# Autodesk Inventor assembly: main'
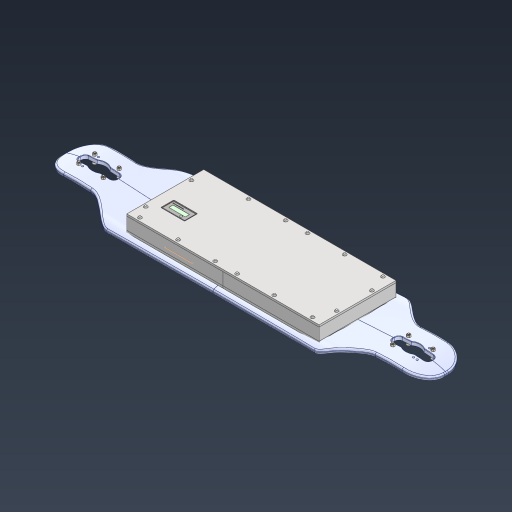
[picture p0: Inventor's stored thumbnail of the model, 512x512]
Saved by Autodesk Inventor 2023 (Build 270158000, 158)
## iProperties
Created: 2025-11-13
Part Number: main'
Document SubType Name: Assembly
Designer: szymo
Author: szymo
## iProperties of the stored document PG7 CABLE GLAND.ipt
Created: 2025-06-09
Part Number: PG7 CABLE GLAND
Material: Generic
Description: STEP AP214
Document SubType Name: Modeling
Designer: szymo
Density: 1 g/cm^3
Appearance: Default
Sending System: SolidWorks 2024
Preprocessor: SwSTEP 2.0
Title: PG7 CABLE GLAND.STEP
Revision Number: ANY
## Documents named in this file (32)
- D:\tech\diy\e-skateboard\projekcik-inventor\main.iam
- D:\tech\diy\e-skateboard\projekcik-inventor\mini-pakiet-12sp1.iam
- D:\tech\diy\e-skateboard\projekcik-inventor\6384 Motor.ipt
- D:\tech\diy\e-skateboard\projekcik-inventor\longboard\Longboard FreeRide.iam
- D:\tech\diy\e-skateboard\projekcik-inventor\vesc42.ipt
- D:\tech\diy\e-skateboard\projekcik-inventor\xt90.iam
- D:\tech\diy\e-skateboard\projekcik-inventor\buttoj\16mm-LED-Power-Button.iam
- **D:\tech\diy\e-skateboard\projekcik-inventor\main.iam*LocalDocs*xAaaaaxaaAaaaaaaaAaaaq0hoRf*PG7 CABLE GLAND.ipt
- D:\tech\diy\e-skateboard\projekcik-inventor\other-parts\deseczka_dol_check - 7.ipt
- D:\tech\diy\e-skateboard\projekcik-inventor\fuse.iam
- D:\tech\diy\e-skateboard\projekcik-inventor\led_buck_conv.ipt
- D:\tech\diy\e-skateboard\projekcik-inventor\battery_status_monitor.iam
- D:\tech\diy\e-skateboard\projekcik-inventor\MKS_express.ipt
- D:\tech\diy\e-skateboard\projekcik-inventor\controller_reveiver.ipt
- D:\tech\diy\e-skateboard\projekcik-inventor\buck_holder.ipt
- D:\tech\diy\e-skateboard\projekcik-inventor\vesc_holder.ipt
- D:\tech\diy\e-skateboard\projekcik-inventor\my_own_pcb.ipt
- D:\tech\diy\e-skateboard\projekcik-inventor\my_pcb_holder.ipt
- D:\tech\diy\e-skateboard\projekcik-inventor\claw_nut.ipt
- D:\tech\diy\e-skateboard\projekcik-inventor\case0.ipt
- D:\tech\diy\e-skateboard\projekcik-inventor\case1.ipt
- D:\tech\diy\e-skateboard\projekcik-inventor\BMS.iam
- D:\tech\diy\e-skateboard\projekcik-inventor\petg_holder.ipt
- D:\tech\diy\e-skateboard\projekcik-inventor\petg_holder_2.ipt
- D:\tech\diy\e-skateboard\projekcik-inventor\other-parts\deseczka_dol_check - 7 second.ipt
- D:\tech\diy\e-skateboard\projekcik-inventor\petg_skeleton_ceil.ipt
- D:\tech\diy\e-skateboard\projekcik-inventor\tpu_ceil.ipt
- D:\tech\diy\e-skateboard\projekcik-inventor\wallet\LedgerX.ipt
- D:\tech\diy\e-skateboard\projekcik-inventor\wallet\mechanical-slim-wallet-1.snapshot.7\wallet v2.ipt
- D:\tech\diy\e-skateboard\projekcik-inventor\kindle.ipt
- D:\tech\diy\e-skateboard\projekcik-inventor\PG7 CABLE GLAND.STEP
- D:\tech\diy\e-skateboard\projekcik-inventor\DIY.step
## Components (62 placed, 29 different names)
1. mini-pakiet-12sp1:1 [sub-assembly] — Mate:1, Flush:11, Flush:12, Tangent:1, Tangent:2, Mate:2
2. mini-pakiet-12sp1:2 [sub-assembly] — Mate:1, Flush:11, Flush:12, Tangent:3
3. 6384 Motor:1
4. Longboard FreeRide:1 [sub-assembly]
5. vesc42:1 — Flush:13, Mate:9, Tangent:4
6. xt90:1 [sub-assembly] — Flush:17, Mate:11, Mate:12
7. 16mm-LED-Power-Button:1 [sub-assembly] — Mate:13, Mate:14
8. PG7 CABLE GLAND:1
9. deseczka_dol_check - 7:1 — Flush:50, Mate:43, Flush:51
10. fuse:1 [sub-assembly] — Tangent:3, Mate:3, Mate:4, Mate:8
11. led_buck_conv:1 — Flush:9
12. battery_status_monitor:1 [sub-assembly] — Mate:45
13. MKS_express:1
14. controller_reveiver:1
15. buck_holder:1 — Flush:9
16. vesc_holder:1 — Flush:13, Mate:10
17. my_own_pcb:1 — Flush:14
18. my_pcb_holder:1 — Flush:14
19. case0:1 — Tangent:1, Tangent:2, Mate:2, Flush:16, Mate:15, Mate:16, Mate:17, Mate:18, Mate:19, Mate:20, Mate:21, Flush:18, Flush:19, Flush:20, Flush:21, Flush:22, Flush:23, Flush:24, Mate:22, Mate:23, Mate:24, Mate:25, Mate:26, Mate:27, Mate:28, Mate:29, Flush:25, Flush:26, Flush:27, Flush:28, Flush:29, Flush:30, Flush:31, Flush:32, Flush:47, Flush:48, Mate:44, Flush:52, Flush:53
20. case1:1 — Flush:16, Mate:3, Mate:4, Mate:6, Mate:7, Mate:10, Flush:17, Mate:11, Mate:13, Mate:14, Mate:30, Mate:31, Mate:32, Mate:33, Mate:34, Mate:35, Mate:36, Mate:37, Mate:38, Mate:39, Mate:40, Mate:41, Flush:33, Flush:34, Flush:35, Flush:36, Flush:37, Flush:38, Flush:39, Flush:40, Flush:41, Flush:42, Flush:43, Flush:44, Flush:45, Flush:46, Mate:42, Flush:49, Flush:50, Mate:43, Flush:51, Flush:54, Flush:55, Flush:56
21. PG7 CABLE GLAND:2
22. PG7 CABLE GLAND:3
23. PG7 CABLE GLAND:4
24. BMS:1 [sub-assembly] — Mate:6, Mate:7, Mate:8, Mate:9, Tangent:4, Mate:12
25. claw_nut:1
26. petg_holder:1 — Flush:45, Flush:46
27. petg_holder_2:1 — Flush:47, Flush:48
28. claw_nut:29 — Mate:42, Flush:49
29. deseczka_dol_check - 7 second:1 — Mate:44, Flush:52, Flush:53
30. petg_skeleton_ceil:1 — Flush:54, Flush:55, Flush:57, Flush:58, Mate:45
31. tpu_ceil:1 — Flush:56, Flush:57, Flush:58
32. LedgerX:1
33. wallet v2:1
34. kindle:1
35. LedgerX:2
36. claw_nut:17 — Mate:30, Flush:38, Angle:2
37. claw_nut:18 — Mate:41, Flush:39, Angle:12
38. claw_nut:19 — Mate:34, Flush:36, Angle:8
39. claw_nut:20 — Mate:40, Flush:42, Angle:9
40. claw_nut:21 — Mate:39, Flush:43, Angle:6
41. claw_nut:22 — Mate:38, Flush:44, Angle:4
42. claw_nut:23 — Mate:37, Flush:41, Angle:1
43. claw_nut:24 — Mate:36, Flush:40, Angle:11
44. claw_nut:25 — Mate:35, Flush:37, Angle:10
45. claw_nut:26 — Mate:33, Flush:35, Angle:7
46. claw_nut:27 — Mate:32, Flush:34, Angle:5
47. claw_nut:28 — Mate:31, Flush:33, Angle:3
48. claw_nut:8 — Mate:20, Flush:18, Angle:15
49. claw_nut:9 — Mate:22, Flush:29, Angle:23
50. claw_nut:10 — Mate:23, Flush:28, Angle:21
51. claw_nut:11 — Mate:24, Flush:30, Angle:25
52. claw_nut:12 — Mate:25, Flush:27, Angle:19
53. claw_nut:13 — Mate:26, Flush:31, Angle:18
54. claw_nut:14 — Mate:27, Flush:26, Angle:16
55. claw_nut:15 — Mate:28, Flush:32, Angle:13
56. claw_nut:16 — Mate:29, Flush:25, Angle:27
57. claw_nut:7 — Mate:21, Flush:24, Angle:14, Angle:27
58. claw_nut:2 — Mate:16, Flush:21, Angle:22
59. claw_nut:3 — Mate:17, Flush:22, Angle:20
60. claw_nut:4 — Mate:15, Flush:20, Angle:24
61. claw_nut:5 — Mate:19, Flush:23, Angle:17
62. claw_nut:6 — Mate:18, Flush:19, Angle:26
## Relationships (124: Flush 48, Mate 45, Angle 27, Tangent 4)
- Flush:9: led_buck_conv:1 ↔ buck_holder:1
- Mate:1 (10 mm): mini-pakiet-12sp1:1 ↔ mini-pakiet-12sp1:2
- Flush:11: mini-pakiet-12sp1:1 ↔ mini-pakiet-12sp1:2
- Flush:12: mini-pakiet-12sp1:1 ↔ mini-pakiet-12sp1:2
- Flush:13: vesc42:1 ↔ vesc_holder:1
- Flush:14: my_own_pcb:1 ↔ my_pcb_holder:1
- Tangent:1 (2 mm): mini-pakiet-12sp1:1 ↔ case0:1
- Tangent:2: mini-pakiet-12sp1:1 ↔ case0:1
- Mate:2: mini-pakiet-12sp1:1 ↔ case0:1
- Flush:16: case0:1 ↔ case1:1
- Tangent:3 (5 mm): mini-pakiet-12sp1:2 ↔ fuse:1
- Mate:3: fuse:1 ↔ case1:1
- Mate:4 (3 mm): fuse:1 ↔ case1:1
- [Mate] (4.15 mm): case1:1 ↔ BMS:1
- Mate:6 (3 mm): case1:1 ↔ BMS:1
- Mate:7: case1:1 ↔ BMS:1
- Mate:8 (5 mm): fuse:1 ↔ BMS:1
- Mate:9 (5 mm): vesc42:1 ↔ BMS:1
- Tangent:4 (3 mm): vesc42:1 ↔ BMS:1
- Mate:10: vesc_holder:1 ↔ case1:1
- Flush:17 (3.5 mm): xt90:1 ↔ case1:1
- Mate:11 (1 mm): xt90:1 ↔ case1:1
- Mate:12 (5 mm): xt90:1 ↔ BMS:1
- Mate:13: 16mm-LED-Power-Button:1 ↔ case1:1
- Mate:14: 16mm-LED-Power-Button:1 ↔ case1:1
- Mate:15: case0:1 ↔ claw_nut:4
- Mate:16: case0:1 ↔ claw_nut:2
- Mate:17: case0:1 ↔ claw_nut:3
- Mate:18: case0:1 ↔ claw_nut:6
- Mate:19: case0:1 ↔ claw_nut:5
- Mate:20: case0:1 ↔ claw_nut:8
- Mate:21: case0:1 ↔ claw_nut:7
- Flush:18: case0:1 ↔ claw_nut:8
- Flush:19: case0:1 ↔ claw_nut:6
- Flush:20: case0:1 ↔ claw_nut:4
- Flush:21: case0:1 ↔ claw_nut:2
- Flush:22: case0:1 ↔ claw_nut:3
- Flush:23: case0:1 ↔ claw_nut:5
- Flush:24: case0:1 ↔ claw_nut:7
- Mate:22: case0:1 ↔ claw_nut:9
- Mate:23: case0:1 ↔ claw_nut:10
- Mate:24: case0:1 ↔ claw_nut:11
- Mate:25: case0:1 ↔ claw_nut:12
- Mate:26: case0:1 ↔ claw_nut:13
- Mate:27: case0:1 ↔ claw_nut:14
- Mate:28: case0:1 ↔ claw_nut:15
- Mate:29: case0:1 ↔ claw_nut:16
- Flush:25: case0:1 ↔ claw_nut:16
- Flush:26: case0:1 ↔ claw_nut:14
- Flush:27: case0:1 ↔ claw_nut:12
- Flush:28: case0:1 ↔ claw_nut:10
- Flush:29: case0:1 ↔ claw_nut:9
- Flush:30: case0:1 ↔ claw_nut:11
- Flush:31: case0:1 ↔ claw_nut:13
- Flush:32: case0:1 ↔ claw_nut:15
- Mate:30: case1:1 ↔ claw_nut:17
- Mate:31: case1:1 ↔ claw_nut:28
- Mate:32: case1:1 ↔ claw_nut:27
- Mate:33: case1:1 ↔ claw_nut:26
- Mate:34: case1:1 ↔ claw_nut:19
- Mate:35: case1:1 ↔ claw_nut:25
- Mate:36: case1:1 ↔ claw_nut:24
- Mate:37: case1:1 ↔ claw_nut:23
- Mate:38: case1:1 ↔ claw_nut:22
- Mate:39: case1:1 ↔ claw_nut:21
- Mate:40: case1:1 ↔ claw_nut:20
- Mate:41: case1:1 ↔ claw_nut:18
- Flush:33: case1:1 ↔ claw_nut:28
- Flush:34: case1:1 ↔ claw_nut:27
- Flush:35: case1:1 ↔ claw_nut:26
- Flush:36: case1:1 ↔ claw_nut:19
- Flush:37: case1:1 ↔ claw_nut:25
- Flush:38: case1:1 ↔ claw_nut:17
- Flush:39: case1:1 ↔ claw_nut:18
- Flush:40: case1:1 ↔ claw_nut:24
- Flush:41: case1:1 ↔ claw_nut:23
- Flush:42: case1:1 ↔ claw_nut:20
- Flush:43: case1:1 ↔ claw_nut:21
- Flush:44: case1:1 ↔ claw_nut:22
- Flush:45: case1:1 ↔ petg_holder:1
- Flush:46: case1:1 ↔ petg_holder:1
- Flush:47: case0:1 ↔ petg_holder_2:1
- Flush:48: case0:1 ↔ petg_holder_2:1
- Mate:42: case1:1 ↔ claw_nut:29
- Flush:49: case1:1 ↔ claw_nut:29
- Flush:50: deseczka_dol_check - 7:1 ↔ case1:1
- Mate:43: deseczka_dol_check - 7:1 ↔ case1:1
- Flush:51: deseczka_dol_check - 7:1 ↔ case1:1
- Mate:44: case0:1 ↔ deseczka_dol_check - 7 second:1
- Flush:52: case0:1 ↔ deseczka_dol_check - 7 second:1
- Flush:53: case0:1 ↔ deseczka_dol_check - 7 second:1
- Flush:54: case1:1 ↔ petg_skeleton_ceil:1
- Flush:55: case1:1 ↔ petg_skeleton_ceil:1
- Flush:56: case1:1 ↔ tpu_ceil:1
- Flush:57: petg_skeleton_ceil:1 ↔ tpu_ceil:1
- Flush:58: petg_skeleton_ceil:1 ↔ tpu_ceil:1
- Angle:1 (0 deg): claw_nut:23
- Angle:2 (0 deg): claw_nut:17
- Angle:3 (0 deg): claw_nut:28
- Angle:4 (0 deg): claw_nut:22
- Angle:5 (0 deg): claw_nut:27
- Angle:6 (0 deg): claw_nut:21
- Angle:7 (0 deg): claw_nut:26
- Angle:8 (0 deg): claw_nut:19
- Angle:9 (0 deg): claw_nut:20
- Angle:10 (0 deg): claw_nut:25
- Angle:11 (0 deg): claw_nut:24
- Angle:12 (0 deg): claw_nut:18
- Angle:13 (0 deg): claw_nut:15
- Angle:14 (0 deg): claw_nut:7
- Angle:15 (0 deg): claw_nut:8
- Angle:16 (0 deg): claw_nut:14
- Angle:17 (0 deg): claw_nut:5
- Angle:18 (0 deg): claw_nut:13
- Angle:19 (0 deg): claw_nut:12
- Angle:20 (0 deg): claw_nut:3
- Angle:21 (0 deg): claw_nut:10
- Angle:22 (0 deg): claw_nut:2
- Angle:23 (0 deg): claw_nut:9
- Angle:24 (0 deg): claw_nut:4
- Angle:25 (0 deg): claw_nut:11
- Angle:26 (0 deg): claw_nut:6
- Mate:45: battery_status_monitor:1 ↔ petg_skeleton_ceil:1
- Angle:27 (0 deg): claw_nut:16 ↔ claw_nut:7
